# Autodesk Inventor assembly: Battery Pack - Samsung 25R -8-8-4
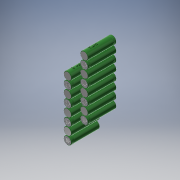
[picture p0: Inventor's stored thumbnail of the model, 180x180]
Saved by Autodesk Inventor 2019.2 (Build 232265000, 265)
## iProperties
Created: 2019-03-02
Part Number: Battery Pack - Samsung 25R -8-8-4
Document SubType Name: Assembly
Designer: Petar
Author: Petar
## Documents named in this file (2)
- D:\OMG\E-Board\CAD\Inventor\Electrical Components\Battery Pack - Samsung 25R -8-8-4.iam
- D:\OMG\E-Board\CAD\Inventor\Electrical Components\Battery Cell - Samsung.ipt
## Components (16 placed, 1 different names)
1. Battery Cell - Samsung:1 — Tangent:1, Flush:1, Flush:2
2. Battery Cell - Samsung:2 — Tangent:1, Flush:1, Flush:2, Tangent:3, Flush:5, Flush:6
3. Battery Cell - Samsung:3 — Tangent:3, Flush:5, Flush:6
4. Battery Cell - Samsung:4 — Tangent:7, Flush:13, Flush:14
5. Battery Cell - Samsung:5 — Tangent:7, Flush:13, Flush:14
6. Battery Cell - Samsung:6
7. Battery Cell - Samsung:7
8. Battery Cell - Samsung:8
9. Battery Cell - Samsung:9
10. Battery Cell - Samsung:10
11. Battery Cell - Samsung:11
12. Battery Cell - Samsung:12
13. Battery Cell - Samsung:13
14. Battery Cell - Samsung:14
15. Battery Cell - Samsung:15
16. Battery Cell - Samsung:16
## Relationships (42: Flush 28, Tangent 14)
- Tangent:1: Battery Cell - Samsung:1 ↔ Battery Cell - Samsung:2
- Flush:1: Battery Cell - Samsung:1 ↔ Battery Cell - Samsung:2
- Flush:2: Battery Cell - Samsung:1 ↔ Battery Cell - Samsung:2
- [Tangent]: Battery Cell - Samsung:3 ↔ Battery Cell - Samsung:4
- [Flush]: Battery Cell - Samsung:3 ↔ Battery Cell - Samsung:4
- [Flush]: Battery Cell - Samsung:3 ↔ Battery Cell - Samsung:4
- Tangent:3: Battery Cell - Samsung:2 ↔ Battery Cell - Samsung:3
- Flush:5: Battery Cell - Samsung:2 ↔ Battery Cell - Samsung:3
- Flush:6: Battery Cell - Samsung:2 ↔ Battery Cell - Samsung:3
- [Tangent]: Battery Cell - Samsung:5 ↔ Battery Cell - Samsung:6
- [Flush]: Battery Cell - Samsung:5 ↔ Battery Cell - Samsung:6
- [Flush]: Battery Cell - Samsung:5 ↔ Battery Cell - Samsung:6
- [Tangent]: Battery Cell - Samsung:7 ↔ Battery Cell - Samsung:8
- [Flush]: Battery Cell - Samsung:7 ↔ Battery Cell - Samsung:8
- [Flush]: Battery Cell - Samsung:7 ↔ Battery Cell - Samsung:8
- [Tangent]: Battery Cell - Samsung:6 ↔ Battery Cell - Samsung:7
- [Flush]: Battery Cell - Samsung:6 ↔ Battery Cell - Samsung:7
- [Flush]: Battery Cell - Samsung:6 ↔ Battery Cell - Samsung:7
- Tangent:7: Battery Cell - Samsung:4 ↔ Battery Cell - Samsung:5
- Flush:13: Battery Cell - Samsung:4 ↔ Battery Cell - Samsung:5
- Flush:14: Battery Cell - Samsung:4 ↔ Battery Cell - Samsung:5
- [Tangent]: Battery Cell - Samsung:9 ↔ Battery Cell - Samsung:10
- [Flush]: Battery Cell - Samsung:9 ↔ Battery Cell - Samsung:10
- [Flush]: Battery Cell - Samsung:9 ↔ Battery Cell - Samsung:10
- [Tangent]: Battery Cell - Samsung:11 ↔ Battery Cell - Samsung:12
- [Flush]: Battery Cell - Samsung:11 ↔ Battery Cell - Samsung:12
- [Flush]: Battery Cell - Samsung:11 ↔ Battery Cell - Samsung:12
- [Tangent]: Battery Cell - Samsung:10 ↔ Battery Cell - Samsung:11
- [Flush]: Battery Cell - Samsung:10 ↔ Battery Cell - Samsung:11
- [Flush]: Battery Cell - Samsung:10 ↔ Battery Cell - Samsung:11
- [Tangent]: Battery Cell - Samsung:13 ↔ Battery Cell - Samsung:14
- [Flush]: Battery Cell - Samsung:13 ↔ Battery Cell - Samsung:14
- [Flush]: Battery Cell - Samsung:13 ↔ Battery Cell - Samsung:14
- [Tangent]: Battery Cell - Samsung:15 ↔ Battery Cell - Samsung:16
- [Flush]: Battery Cell - Samsung:15 ↔ Battery Cell - Samsung:16
- [Flush]: Battery Cell - Samsung:15 ↔ Battery Cell - Samsung:16
- [Tangent]: Battery Cell - Samsung:14 ↔ Battery Cell - Samsung:15
- [Flush]: Battery Cell - Samsung:14 ↔ Battery Cell - Samsung:15
- [Flush]: Battery Cell - Samsung:14 ↔ Battery Cell - Samsung:15
- [Tangent]: Battery Cell - Samsung:12 ↔ Battery Cell - Samsung:13
- [Flush]: Battery Cell - Samsung:12 ↔ Battery Cell - Samsung:13
- [Flush]: Battery Cell - Samsung:12 ↔ Battery Cell - Samsung:13
## Named parameters: d4_d1 = 0 mm, d5_d3 = 0 mm, d6_d0 = 0 mm, d10_d1 = 0 mm, d11_d3 = 0 mm, d12_d4_d1 = 0 mm, d13_d5_d3 = 0 mm, d14_d6_d0 = 0 mm, d15_d7 = 0 mm, d16_d8 = 0 mm, d17_d9 = 0 mm, d18_d0 = 0 mm, d58_d9 = 0 mm, d59_d10_d1 = 0 mm, d60_d11_d3 = 0 mm, d61_d12_d4_d1 = 0 mm, d62_d13_d5_d3 = 0 mm, d63_d14_d6_d0 = 0 mm, d64_d15_d7 = 0 mm, d65_d16_d8 = 0 mm, d66_d17_d9 = 0 mm, d67_d18_d0 = 0 mm, d68_d19 = 0 mm, d69_d20 = 0 mm, d70_d21 = 0 mm, d71_d0 = 0 mm, d72_d1 = 0 mm, d73_d3 = 0 mm, d74_d4_d1 = 0 mm, d75_d5_d3 = 0 mm, d76_d6_d0 = 0 mm, d77_d7 = 0 mm, d78_d8 = 0 mm
